# Autodesk Inventor assembly: Cam_DespLP
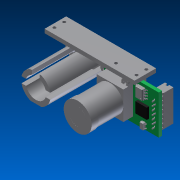
[picture p0: Inventor's stored thumbnail of the model, 180x180]
Saved by Autodesk Inventor 2012 (Build 160160000, 160)
## iProperties
Created: 2015-11-18
Part Number: Cam_DespLP
Document SubType Name: Assembly
Designer: Alex Becerra
Mass: 16.1208 g
Surface Area: 93.049 cm^2
Volume: 6.16795 cm^3
Density: 2.61364 g/cm^3
Author: Alex Becerra
## Documents named in this file (3)
- C:\Users\Thinkpad\Cubesat SUChAI\Mecanica\Modelo_3D\Placa_payloads\Cam_DespLP\Cam_DespLP.iam
- C:\Users\Thinkpad\Cubesat SUChAI\Mecanica\Modelo_3D\Placa_payloads\Camara\Camara_final.iam
- C:\Users\Thinkpad\Cubesat SUChAI\Mecanica\Modelo_3D\Placa_payloads\Lanzamiento_LP\Imported Components\Despliegue3\Despliegue3.ipt
## Components (2 placed, 2 different names)
1. Camara_final:1 [sub-assembly] — Mate:1, Mate:2
2. Despliegue3:1 — Mate:1, Mate:2
## Relationships (2: Mate 2)
- Mate:1: Camara_final:1 ↔ Despliegue3:1
- Mate:2: Camara_final:1 ↔ Despliegue3:1
